# Autodesk Inventor assembly: POM_T5_14
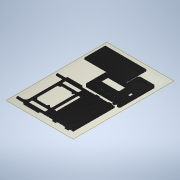
[picture p0: Inventor's stored thumbnail of the model, 180x180]
Saved by Autodesk Inventor 2020 (Build 240168000, 168)
## iProperties
Created: 2021-08-27
Part Number: POM_T5_14
Document SubType Name: Assembly
Designer: Masato
Author: Masato
## Documents named in this file (7)
- C:\Inventor\SUSTAINA-OP\Cam\POM_T5_14.iam
- C:\Inventor\SUSTAINA-OP\Cam\DisposableBoard.ipt
- C:\Inventor\SUSTAINA-OP\UpperBody\Cockpit\Cockpit_carrier_board_frame.ipt
- C:\Inventor\SUSTAINA-OP\UpperBody\Cockpit\Cockpit_battery_bottom_frame.ipt
- C:\Inventor\SUSTAINA-OP\UpperBody\Cockpit\Cockpit_battery_front_frame.ipt
- C:\Inventor\SUSTAINA-OP\UpperBody\Cockpit\Cockpit_front_frame.ipt
- C:\Inventor\SUSTAINA-OP\UpperBody\Cockpit\Cockpit_side_frame_MIR.ipt
## Components (6 placed, 6 different names)
1. DisposableBoard:1 — メイト:2, メイト:1, フラッシュ:1, フラッシュ:2, メイト:4, メイト:5, メイト:6, フラッシュ:3, フラッシュ:4, メイト:9, フラッシュ:7, メイト:11, フラッシュ:9, フラッシュ:10
2. Cockpit_carrier_board_frame:1 — メイト:4, フラッシュ:3, フラッシュ:4, メイト:7, フラッシュ:5, フラッシュ:8
3. Cockpit_battery_bottom_frame:1 — メイト:5, メイト:7, フラッシュ:5, メイト:8
4. Cockpit_battery_front_frame:1 — メイト:6, メイト:8, メイト:10, フラッシュ:10
5. Cockpit_front_frame:1 — メイト:11, フラッシュ:8, フラッシュ:9
6. Cockpit_side_frame_MIR:1 — メイト:9, フラッシュ:7, メイト:10
## Relationships (19: Mate 10, Flush 9)
- メイト:2 [Mate]: DisposableBoard:1
- メイト:1 [Mate]: DisposableBoard:1
- フラッシュ:1 [Flush]: DisposableBoard:1
- フラッシュ:2 [Flush]: DisposableBoard:1
- メイト:4 [Mate]: DisposableBoard:1 ↔ Cockpit_carrier_board_frame:1
- メイト:5 [Mate]: DisposableBoard:1 ↔ Cockpit_battery_bottom_frame:1
- メイト:6 [Mate]: DisposableBoard:1 ↔ Cockpit_battery_front_frame:1
- フラッシュ:3 [Flush] (2 mm): DisposableBoard:1 ↔ Cockpit_carrier_board_frame:1
- フラッシュ:4 [Flush] (2 mm): DisposableBoard:1 ↔ Cockpit_carrier_board_frame:1
- メイト:7 [Mate] (2.5 mm): Cockpit_carrier_board_frame:1 ↔ Cockpit_battery_bottom_frame:1
- フラッシュ:5 [Flush]: Cockpit_carrier_board_frame:1 ↔ Cockpit_battery_bottom_frame:1
- メイト:8 [Mate] (2.5 mm): Cockpit_battery_bottom_frame:1 ↔ Cockpit_battery_front_frame:1
- メイト:9 [Mate]: DisposableBoard:1 ↔ Cockpit_side_frame_MIR:1
- フラッシュ:7 [Flush] (2 mm): DisposableBoard:1 ↔ Cockpit_side_frame_MIR:1
- メイト:10 [Mate] (2.25 mm): Cockpit_battery_front_frame:1 ↔ Cockpit_side_frame_MIR:1
- メイト:11 [Mate]: DisposableBoard:1 ↔ Cockpit_front_frame:1
- フラッシュ:8 [Flush]: Cockpit_carrier_board_frame:1 ↔ Cockpit_front_frame:1
- フラッシュ:9 [Flush] (2 mm): DisposableBoard:1 ↔ Cockpit_front_frame:1
- フラッシュ:10 [Flush] (1.5 mm): DisposableBoard:1 ↔ Cockpit_battery_front_frame:1
